# Autodesk Inventor assembly: sus-target-with-W
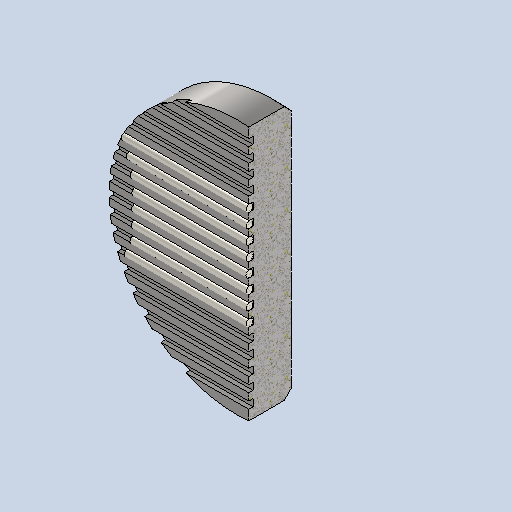
[picture p0: Inventor's stored thumbnail of the model, 512x512]
Saved by Autodesk Inventor 2026 (Build 300175050, 175E)
## iProperties
Created: 2025-08-20
Part Number: sus-target-with-W
Document SubType Name: Assembly
Designer: kuzmin
Author: kuzmin
## Documents named in this file (3)
- C:\Users\queez\Dropbox\Drawings\PIHTI\Plasma Vessel\Boron-Target\sus-target-with-W.iam
- C:\Users\queez\Dropbox\Drawings\PIHTI\Plasma Vessel\Boron-Target\boron-target-grooved.ipt
- C:\Users\queez\Dropbox\Drawings\PIHTI\Plasma Vessel\Boron-Target\w-wire-10.ipt
## Components (9 placed, 2 different names)
1. boron-target-grooved:1 — Tangent:1, Tangent:2, Tangent:3, Tangent:4, Tangent:5, Tangent:6, Tangent:7, Tangent:8, Tangent:9, Tangent:10, Tangent:11, Tangent:12, Tangent:13, Tangent:14, Tangent:15, Tangent:16
2. w-wire-10:1 — Tangent:1, Tangent:2
3. w-wire-10:2 — Tangent:5, Tangent:6
4. w-wire-10:3 — Tangent:3, Tangent:4
5. w-wire-10:4 — Tangent:11, Tangent:16
6. w-wire-10:5 — Tangent:7, Tangent:8
7. w-wire-10:6 — Tangent:9, Tangent:10
8. w-wire-10:7 — Tangent:12, Tangent:13
9. w-wire-10:8 — Tangent:14, Tangent:15
## Relationships (16: Tangent 16)
- Tangent:1: boron-target-grooved:1 ↔ w-wire-10:1
- Tangent:2: boron-target-grooved:1 ↔ w-wire-10:1
- Tangent:3: boron-target-grooved:1 ↔ w-wire-10:3
- Tangent:4: boron-target-grooved:1 ↔ w-wire-10:3
- Tangent:5: boron-target-grooved:1 ↔ w-wire-10:2
- Tangent:6: boron-target-grooved:1 ↔ w-wire-10:2
- Tangent:7: boron-target-grooved:1 ↔ w-wire-10:5
- Tangent:8: boron-target-grooved:1 ↔ w-wire-10:5
- Tangent:9: boron-target-grooved:1 ↔ w-wire-10:6
- Tangent:10: boron-target-grooved:1 ↔ w-wire-10:6
- Tangent:11: boron-target-grooved:1 ↔ w-wire-10:4
- Tangent:12: boron-target-grooved:1 ↔ w-wire-10:7
- Tangent:13: boron-target-grooved:1 ↔ w-wire-10:7
- Tangent:14: boron-target-grooved:1 ↔ w-wire-10:8
- Tangent:15: boron-target-grooved:1 ↔ w-wire-10:8
- Tangent:16: boron-target-grooved:1 ↔ w-wire-10:4
